# Autodesk Inventor assembly: Full House
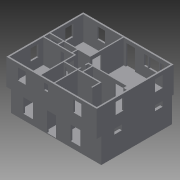
[picture p0: Inventor's stored thumbnail of the model, 180x180]
Saved by Autodesk Inventor 2013 (Build 170138000, 138)
## iProperties
Created: 2013-06-17
Part Number: Full House
Document SubType Name: Assembly
Designer: Joey
Author: Joey
## Documents named in this file (3)
- C:\Users\Joey\Documents\NIST\57th Avenue House\Full House.iam
- C:\Users\Joey\Documents\NIST\57th Avenue House\Basement.ipt
- C:\Users\Joey\Documents\NIST\57th Avenue House\First Floor.ipt
## Components (2 placed, 2 different names)
1. Basement:1 — Flush:1, Flush:2, Mate:1
2. First Floor:1 — Flush:1, Flush:2, Mate:1
## Relationships (3: Flush 2, Mate 1)
- Flush:1: Basement:1 ↔ First Floor:1
- Flush:2 (-152.4 mm): Basement:1 ↔ First Floor:1
- Mate:1: Basement:1 ↔ First Floor:1
